# Autodesk Inventor assembly: TAZ 6 Plate Convex Model
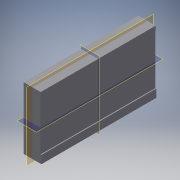
[picture p0: Inventor's stored thumbnail of the model, 180x180]
Saved by Autodesk Inventor 2019 (Build 230136000, 136)
## iProperties
Created: 2021-05-14
Part Number: TAZ 6 Plate Convex Model
Document SubType Name: Assembly
Designer: Eric
Author: Eric
## Documents named in this file (4)
- C:\Users\Eric\Documents\! - Uni\Year 4\MENG-Robot-Fab-Project\Models\For_Optimiser\Static Parts Assembly\TAZ 6 Assembly\TAZ 6 Plate Convex Model.iam
- C:\Users\Eric\Documents\! - Uni\Year 4\MENG-Robot-Fab-Project\Models\For_Optimiser\Static Parts Assembly\TAZ 6 Assembly\TAZ6Plate_1.ipt
- C:\Users\Eric\Documents\! - Uni\Year 4\MENG-Robot-Fab-Project\Models\For_Optimiser\Static Parts Assembly\TAZ 6 Assembly\TAZ6Plate_2.ipt
- C:\Users\Eric\Documents\! - Uni\Year 4\MENG-Robot-Fab-Project\Models\For_Optimiser\Static Parts Assembly\TAZ 6 Assembly\TAZ6Plate_3.ipt
## Components (3 placed, 3 different names)
1. TAZ6Plate_1:1 — Symmetry:1, Symmetry:2, Symmetry:3
2. TAZ6Plate_2:1
3. TAZ6Plate_3:1 — Symmetry:1, Symmetry:2, Symmetry:3
## Relationships (3: Symmetry 3)
- Symmetry:1: TAZ6Plate_1:1 ↔ TAZ6Plate_3:1
- Symmetry:2: TAZ6Plate_1:1 ↔ TAZ6Plate_3:1
- Symmetry:3: TAZ6Plate_1:1 ↔ TAZ6Plate_3:1
